# Autodesk Inventor assembly: Assembly1
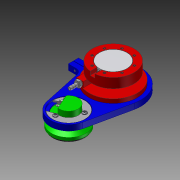
[picture p0: Inventor's stored thumbnail of the model, 180x180]
Saved by Autodesk Inventor 2012 SP1 (Build 160190100, 190)
## iProperties
Created: 2010-02-10
Part Number: Assembly1
Document SubType Name: Assembly
Designer: rconnaug
Author: rconnaug
## Documents named in this file (20)
- D:\Users\ding42\Dropbox\Inventor files\CMS\Module Assembly Station\Gantry\NewGantryParts\OriginalUCSB\ToolHolder\ToolHolder.iam
- D:\Users\ding42\Dropbox\Inventor files\CMS\Module Assembly Station\Gantry\NewGantryParts\OriginalUCSB\ToolHolder\HoseBarbAddOn.ipt
- D:\Users\ding42\Dropbox\Inventor files\CMS\Module Assembly Station\Gantry\NewGantryParts\OriginalUCSB\ToolHolder\ToolHolderSpool.ipt
- D:\Users\ding42\Dropbox\Inventor files\CMS\Module Assembly Station\Gantry\NewGantryParts\OriginalUCSB\ToolHolder\DispenserHolderArm.ipt
- D:\Users\ding42\Dropbox\Inventor files\CMS\Module Assembly Station\Gantry\NewGantryParts\OriginalUCSB\ToolHolder\DispenserHolder.ipt
- D:\Users\ding42\Dropbox\Inventor files\CMS\Module Assembly Station\Gantry\NewGantryParts\OriginalUCSB\ToolHolder\DispenserHolderCapturePlate.ipt
- D:\Users\ding42\Dropbox\Inventor files\CMS\Module Assembly Station\Gantry\NewGantryParts\OriginalUCSB\ToolHolder\BallBearingBall.ipt
- D:\Users\ding42\Dropbox\Inventor files\CMS\Module Assembly Station\Gantry\NewGantryParts\OriginalUCSB\ToolHolder\ContactPuck.ipt
- D:\Users\ding42\Dropbox\Inventor files\CMS\Module Assembly Station\Gantry\NewGantryParts\OriginalUCSB\ToolHolder\5454K740_0.0625ID_Tube_Barb.ipt
- D:\Users\ding42\Dropbox\Inventor files\CMS\Module Assembly Station\Gantry\NewGantryParts\OriginalUCSB\ToolHolder\ToolHolderSlug Body.ipt
- D:\Users\ding42\Dropbox\Inventor files\CMS\Module Assembly Station\Gantry\NewGantryParts\OriginalUCSB\ToolHolder\5454K63_0.125ID_Tube_Barb.ipt
- D:\Users\ding42\Dropbox\Inventor files\CMS\Module Assembly Station\Gantry\NewGantryParts\OriginalUCSB\ToolHolder\91772A030.ipt
- D:\Users\ding42\Dropbox\Inventor files\CMS\Module Assembly Station\Gantry\NewGantryParts\OriginalUCSB\ToolHolder\91251A831.ipt
- D:\Users\ding42\Dropbox\Inventor files\CMS\Module Assembly Station\Gantry\NewGantryParts\OriginalUCSB\ToolHolder\9396K153 Silicone O-Ring .ipt
- D:\Users\ding42\Dropbox\Inventor files\CMS\Module Assembly Station\Gantry\NewGantryParts\OriginalUCSB\ToolHolder\9396K27 Silicone O-Ring.ipt
- D:\Users\ding42\Dropbox\Inventor files\CMS\Module Assembly Station\Gantry\NewGantryParts\OriginalUCSB\ToolHolder\9452K15 Buna-N O-Ring .ipt
- D:\Users\ding42\Dropbox\Inventor files\CMS\Module Assembly Station\Gantry\NewGantryParts\OriginalUCSB\ToolHolder\KSR MicroSwitch.ipt
- D:\Users\ding42\Dropbox\Inventor files\CMS\Module Assembly Station\Gantry\NewGantryParts\OriginalUCSB\ToolHolder\Rolling bearing 51105 GB_T 301-1995.ipt
- D:\Users\ding42\Dropbox\Inventor files\CMS\Module Assembly Station\Gantry\NewGantryParts\OriginalUCSB\ToolHolder\9452K87 Buna-N O-Ring.ipt
- D:\Users\ding42\Dropbox\Inventor files\CMS\Module Assembly Station\Gantry\NewGantryParts\OriginalUCSB\ToolHolder\9452K14 Buna-N O-Ring.ipt
## Components (26 placed, 19 different names)
1. ToolHolderSpool:1 — Mate:2, Mate:1, Mate:3, Flush:1, Mate:9, Mate:10, Angle:3, Angle:4, Mate:12, Flush:4, Mate:16, Angle:5, Angle:7, Insert:8, Mate:24, Tangent:2, Mate:25, Mate:30, Mate:31
2. HoseBarbAddOn:1 — Mate:9, Mate:10, Angle:3, Insert:1
3. ToolHolderSlug Body:1 — Mate:2, Mate:1, Mate:19, Mate:20, Mate:21, Mate:22, Mate:23, Tangent:1, Insert:11
4. DispenserHolderArm:1 — Mate:3, Flush:1, Mate:4, Insert:7, Insert:14
5. DispenserHolder:1 — Mate:4, Mate:7, Mate:8, Insert:2, Insert:3, Insert:12, Insert:13, Insert:15
6. DispenserHolderCapturePlate:1 — Mate:7, Mate:8, Insert:4, Insert:5, Insert:6, Insert:14, Insert:15
7. ContactPuck:1 — Angle:4, Mate:12, Mate:25, Mate:26, Mate:27
8. Rolling bearing GB/T 301-1995 Type 51000 51105:1 — Mate:31, Mate:32
9. BallBearingBall:1 — Flush:4, Mate:16, Mate:17, Mate:18
10. BallBearingBall:2 — Mate:17, Mate:19, Angle:5, Mate:21, Mate:32
11. BallBearingBall:3 — Mate:18, Angle:7, Mate:20, Mate:22, Tangent:3
12. 5454K63_0.125ID_Tube_Barb:1 — Insert:1
13. 5454K740_0.0625ID_Tube_Barb:1 — Insert:2
14. 5454K740_0.0625ID_Tube_Barb:2 — Insert:3
15. 5454K740_0.0625ID_Tube_Barb:3 — Mate:23, Tangent:1
16. 91772A030:1 — Insert:4
17. 91772A030:2 — Insert:6
18. 91772A030:3 — Insert:5
19. 91251A831:1 — Insert:7
20. 9452K87 Buna-N O-Ring:1 — Insert:13
21. 9452K14 Buna-N O-Ring:1 — Insert:12
22. 9396K153 Silicone O-Ring :1 — Insert:8
23. 9396K27 Silicone O-Ring:1 — Mate:24, Tangent:2
24. 9452K15 Buna-N O-Ring :1 — Insert:11
25. KSR MicroSwitch:1 — Mate:26, Mate:28, Flush:5
26. KSR MicroSwitch:2 — Mate:27, Mate:28, Flush:5, Mate:29, Flush:6
## Relationships (53: Mate 26, Insert 13, Angle 7, Flush 4, Tangent 3)
- Mate:2: ToolHolderSpool:1 ↔ ToolHolderSlug Body:1
- Mate:1: ToolHolderSpool:1 ↔ ToolHolderSlug Body:1
- [Angle] (180 deg): ToolHolderSpool:1 ↔ ToolHolderSlug Body:1
- Mate:3: ToolHolderSpool:1 ↔ DispenserHolderArm:1
- Flush:1: ToolHolderSpool:1 ↔ DispenserHolderArm:1
- Mate:4: DispenserHolderArm:1 ↔ DispenserHolder:1
- Mate:7: DispenserHolder:1 ↔ DispenserHolderCapturePlate:1
- Mate:8: DispenserHolder:1 ↔ DispenserHolderCapturePlate:1
- [Angle] (-90 deg): ToolHolderSpool:1 ↔ DispenserHolderArm:1
- Mate:9: ToolHolderSpool:1 ↔ HoseBarbAddOn:1
- Mate:10: ToolHolderSpool:1 ↔ HoseBarbAddOn:1
- Angle:3 (0 deg): ToolHolderSpool:1 ↔ HoseBarbAddOn:1
- Angle:4 (0 deg): ToolHolderSpool:1 ↔ ContactPuck:1
- Mate:12: ToolHolderSpool:1 ↔ ContactPuck:1
- Flush:4: ToolHolderSpool:1 ↔ BallBearingBall:1
- Mate:16 (16.7938 mm): ToolHolderSpool:1 ↔ BallBearingBall:1
- Mate:17: BallBearingBall:1 ↔ BallBearingBall:2
- Mate:18: BallBearingBall:1 ↔ BallBearingBall:3
- Mate:19 (16.7938 mm): ToolHolderSlug Body:1 ↔ BallBearingBall:2
- Angle:5 (60 deg): ToolHolderSpool:1 ↔ BallBearingBall:2
- Angle:7 (30 deg): ToolHolderSpool:1 ↔ BallBearingBall:3
- Mate:20 (-16.7938 mm): ToolHolderSlug Body:1 ↔ BallBearingBall:3
- Mate:21: ToolHolderSlug Body:1 ↔ BallBearingBall:2
- Mate:22: ToolHolderSlug Body:1 ↔ BallBearingBall:3
- Insert:1: HoseBarbAddOn:1 ↔ 5454K63_0.125ID_Tube_Barb:1
- Insert:2: DispenserHolder:1 ↔ 5454K740_0.0625ID_Tube_Barb:1
- Insert:3: DispenserHolder:1 ↔ 5454K740_0.0625ID_Tube_Barb:2
- Mate:23: ToolHolderSlug Body:1 ↔ 5454K740_0.0625ID_Tube_Barb:3
- Tangent:1: ToolHolderSlug Body:1 ↔ 5454K740_0.0625ID_Tube_Barb:3
- Insert:4: DispenserHolderCapturePlate:1 ↔ 91772A030:1
- Insert:5: DispenserHolderCapturePlate:1 ↔ 91772A030:3
- Insert:6: DispenserHolderCapturePlate:1 ↔ 91772A030:2
- Insert:7: DispenserHolderArm:1 ↔ 91251A831:1
- Insert:8: ToolHolderSpool:1 ↔ 9396K153 Silicone O-Ring :1
- Mate:24: ToolHolderSpool:1 ↔ 9396K27 Silicone O-Ring:1
- Tangent:2: ToolHolderSpool:1 ↔ 9396K27 Silicone O-Ring:1
- Insert:11: ToolHolderSlug Body:1 ↔ 9452K15 Buna-N O-Ring :1
- Mate:25: ToolHolderSpool:1 ↔ ContactPuck:1
- Mate:26 (0.0762 mm): ContactPuck:1 ↔ KSR MicroSwitch:1
- Mate:27 (0.127 mm): ContactPuck:1 ↔ KSR MicroSwitch:2
- Mate:28: KSR MicroSwitch:1 ↔ KSR MicroSwitch:2
- Flush:5: KSR MicroSwitch:1 ↔ KSR MicroSwitch:2
- Mate:29: KSR MicroSwitch:2
- Flush:6 (-2 mm): KSR MicroSwitch:2
- Angle:8 (0 deg)
- Tangent:3: BallBearingBall:3
- Mate:30 (0.7 mm): ToolHolderSpool:1
- Mate:31: ToolHolderSpool:1 ↔ Rolling bearing GB/T 301-1995 Type 51000 51105:1
- Mate:32 (-5.48 mm): Rolling bearing GB/T 301-1995 Type 51000 51105:1 ↔ BallBearingBall:2
- Insert:12: DispenserHolder:1 ↔ 9452K14 Buna-N O-Ring:1
- Insert:13: DispenserHolder:1 ↔ 9452K87 Buna-N O-Ring:1
- Insert:14: DispenserHolderArm:1 ↔ DispenserHolderCapturePlate:1
- Insert:15: DispenserHolder:1 ↔ DispenserHolderCapturePlate:1
